# Autodesk Inventor assembly: Dosing
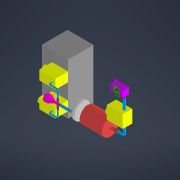
[picture p0: Inventor's stored thumbnail of the model, 180x180]
Saved by Autodesk Inventor 2022 (Build 260153070, 153G)
## iProperties
Created: 2021-07-20
Part Number: Dosing
Document SubType Name: Assembly
Designer: Eakawit_kor
Author: Eakawit_kor
## Documents named in this file (12)
- C:\Users\Eakawit_kor\OneDrive - EASTWATER GROUP\Workspace\5_UUTurbidity\UUTurbidity\1_Hardware\Assembly\Dosing.iam
- C:\Users\Eakawit_kor\OneDrive - EASTWATER GROUP\Workspace\5_UUTurbidity\UUTurbidity\1_Hardware\Part\Reactor.ipt
- C:\Users\Eakawit_kor\OneDrive - EASTWATER GROUP\Workspace\5_UUTurbidity\UUTurbidity\1_Hardware\Part\TopReactor.ipt
- C:\Users\Eakawit_kor\OneDrive - EASTWATER GROUP\Workspace\5_UUTurbidity\UUTurbidity\1_Hardware\Part\BoxChem.ipt
- C:\Users\Eakawit_kor\OneDrive - EASTWATER GROUP\Workspace\5_UUTurbidity\UUTurbidity\1_Hardware\Part\Chemmix.ipt
- C:\Users\Eakawit_kor\OneDrive - EASTWATER GROUP\Workspace\5_UUTurbidity\UUTurbidity\1_Hardware\Part\Mesurement.ipt
- C:\Users\Eakawit_kor\OneDrive - EASTWATER GROUP\Workspace\5_UUTurbidity\UUTurbidity\1_Hardware\PartHelping\Pipe1.ipt
- C:\Users\Eakawit_kor\OneDrive - EASTWATER GROUP\Workspace\5_UUTurbidity\UUTurbidity\1_Hardware\PartHelping\Pipe2.ipt
- C:\Users\Eakawit_kor\OneDrive - EASTWATER GROUP\Workspace\5_UUTurbidity\UUTurbidity\1_Hardware\PartHelping\Pipe3.ipt
- C:\Users\Eakawit_kor\OneDrive - EASTWATER GROUP\Workspace\5_UUTurbidity\UUTurbidity\1_Hardware\PartHelping\SolidnoidV.ipt
- C:\Users\Eakawit_kor\OneDrive - EASTWATER GROUP\Workspace\5_UUTurbidity\UUTurbidity\1_Hardware\PartHelping\Pipe4.ipt
- C:\Users\Eakawit_kor\OneDrive - EASTWATER GROUP\Workspace\5_UUTurbidity\UUTurbidity\2_Electonic\PCB\US001_UUTurbidity.ipt
## Components (14 placed, 11 different names)
1. Reactor:1 — Insert:1, Insert:5
2. TopReactor:1 — Insert:1, Angle:1, Mate:18, Mate:20, Mate:21
3. BoxChem:1 — Angle:1, Mate:4, Angle:2, Angle:3, Mate:13
4. Chemmix:1 — Mate:3, Insert:4, Mate:10, Mate:18, Mate:19, Mate:22
5. Mesurement:1 — Mate:1, Mate:2, Flush:2, Angle:2, Angle:3, Mate:5, Mate:6, Angle:4, Mate:16, Mate:17
6. Pipe1:1 — Mate:3, Mate:8, Mate:10, Mate:11
7. Pipe2:1 — Mate:4, Insert:4, Mate:9, Mate:12
8. Pipe3:1 — Insert:5, Mate:5, Mate:7
9. SolidnoidV:1 — Mate:6, Angle:4, Mate:7, Mate:14, Mate:15
10. SolidnoidV:2 — Mate:9, Flush:3, Mate:12, Mate:13
11. SolidnoidV:3 — Mate:8, Flush:3, Mate:11
12. Pipe4:1 — Mate:14, Mate:15, Mate:16
13. US001_UUTurbidity:1 — Mate:17
14. Pipe4:2 — Mate:19, Mate:20, Mate:21, Mate:22
## Relationships (31: Mate 22, Angle 4, Insert 3, Flush 2)
- Insert:1 (20 mm): Reactor:1 ↔ TopReactor:1
- Mate:1: Mesurement:1
- Mate:2: Mesurement:1
- Flush:2: Mesurement:1
- Angle:1 (180 deg): TopReactor:1 ↔ BoxChem:1
- Mate:3: Chemmix:1 ↔ Pipe1:1
- Mate:4: BoxChem:1 ↔ Pipe2:1
- Insert:4: Chemmix:1 ↔ Pipe2:1
- Angle:2 (0 deg): BoxChem:1 ↔ Mesurement:1
- Angle:3 (180 deg): BoxChem:1 ↔ Mesurement:1
- Insert:5: Reactor:1 ↔ Pipe3:1
- Mate:5: Mesurement:1 ↔ Pipe3:1
- Mate:6: Mesurement:1 ↔ SolidnoidV:1
- Angle:4 (0 deg): Mesurement:1 ↔ SolidnoidV:1
- Mate:7: Pipe3:1 ↔ SolidnoidV:1
- Mate:8: Pipe1:1 ↔ SolidnoidV:3
- Mate:9: Pipe2:1 ↔ SolidnoidV:2
- Flush:3: SolidnoidV:2 ↔ SolidnoidV:3
- Mate:10: Chemmix:1 ↔ Pipe1:1
- Mate:11: Pipe1:1 ↔ SolidnoidV:3
- Mate:12: Pipe2:1 ↔ SolidnoidV:2
- Mate:13: BoxChem:1 ↔ SolidnoidV:2
- Mate:14: SolidnoidV:1 ↔ Pipe4:1
- Mate:15: SolidnoidV:1 ↔ Pipe4:1
- Mate:16: Mesurement:1 ↔ Pipe4:1
- Mate:17: Mesurement:1 ↔ US001_UUTurbidity:1
- Mate:18: TopReactor:1 ↔ Chemmix:1
- Mate:19: Chemmix:1 ↔ Pipe4:2
- Mate:20: TopReactor:1 ↔ Pipe4:2
- Mate:21: TopReactor:1 ↔ Pipe4:2
- Mate:22: Chemmix:1 ↔ Pipe4:2
